# Autodesk Inventor assembly: XY Joint Left
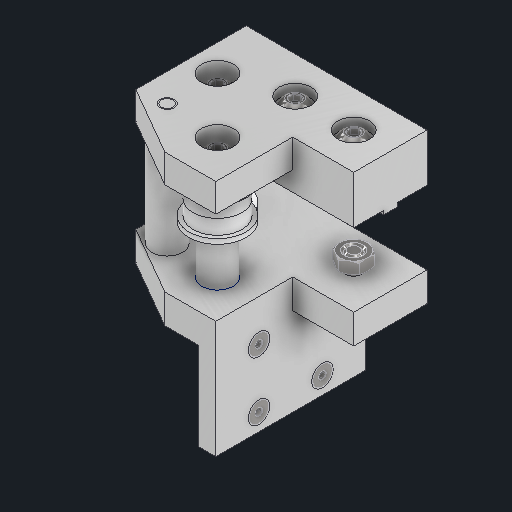
[picture p0: Inventor's stored thumbnail of the model, 512x512]
Saved by Autodesk Inventor 2025.1 (Build 291241020, 241B)
## iProperties
Created: 2025-05-09
Part Number: XY Joint Left
Document SubType Name: Assembly
Designer: AdminForWorker
Title: XY Joint Left
Author: AdminForWorker
## Documents named in this file (10)
- C:\Users\Joshua Eah\Documents\Voron 0.2\CAD\Master Assembly\XY Joint Left.iam
- C:\Users\Joshua Eah\Documents\Voron 0.2\CAD\Machined Parts\XY Joints\XY Joint Left\XY Joint Left.iam
- XY Joint Left.iam
- C:\Users\Joshua Eah\Documents\Voron 0.2\CAD\Master Assembly\F623 Stack.iam
- C:\Users\Joshua Eah\Documents\Voron 0.2\CAD\Master Assembly\Washers (3).iam
- C:\Users\Joshua Eah\Documents\Voron 0.2\CAD\Master Assembly\Hardware\M3 Hexnut.ipt
- C:\Users\Joshua Eah\Documents\Voron 0.2\CAD\Master Assembly\Hardware\M3x25 BHCS.ipt
- C:\Users\Joshua Eah\Documents\Voron 0.2\CAD\Master Assembly\Hardware\M2x6 FHCS.ipt
- C:\Users\Joshua Eah\Documents\Voron 0.2\CAD\Master Assembly\Hardware\M3x12 BHCS.ipt
- C:\Users\Joshua Eah\Documents\Voron 0.2\CAD\Master Assembly\Hardware\M3x6 BHCS.ipt
## Components (16 placed, 8 different names)
1. XY Joint Left:1 [sub-assembly]
2. F623 Stack:2 [sub-assembly]
3. F623 Stack:1 [sub-assembly]
4. Washers (3):1 [sub-assembly]
5. M3 Hexnut:1
6. M3 Hexnut:2
7. M3 Hexnut:3
8. M3x25 BHCS:1
9. M2x6 FHCS:1
10. M2x6 FHCS:2
11. M2x6 FHCS:3
12. M2x6 FHCS:4
13. M3x25 BHCS:2
14. M3x12 BHCS:1
15. M3x12 BHCS:2
16. M3x6 BHCS:1
## Relationships (1: Insert 1)
- [Insert]: XY Joint Left:1 ↔ M3x12 BHCS:1
